# Autodesk Inventor assembly: Lath
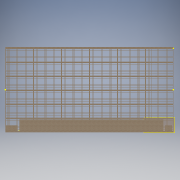
[picture p0: Inventor's stored thumbnail of the model, 180x180]
Saved by Autodesk Inventor 2018 (Build 220112000, 112)
## iProperties
Created: 2019-05-10
Part Number: Lath
Document SubType Name: Assembly
Designer: 10043883
Author: 10043883
## Documents named in this file (5)
- C:\Users\10043883\Documents\GitHub\IED-files\Lathhouse\Lath.iam
- C:\Users\10043883\Documents\GitHub\IED-files\Lathhouse\Lathhouse wall.ipt
- C:\Users\10043883\Documents\GitHub\IED-files\Lathhouse\Foor.ipt
- C:\Users\10043883\Documents\GitHub\IED-files\Lathhouse\Lathhouse roof.ipt
- C:\Users\10043883\Documents\GitHub\IED-files\Lathhouse\Front door.ipt
## Components (5 placed, 4 different names)
1. Foor:1 — Mate:13
2. Lathhouse wall:1 — Mate:11, Mate:12
3. Lathhouse roof:1 — Mate:9, Mate:11
4. Front door:1 — Mate:9
5. Front door:2 — Mate:12, Mate:13
## Relationships (4: Mate 4)
- Mate:9: Lathhouse roof:1 ↔ Front door:1
- Mate:11: Lathhouse wall:1 ↔ Lathhouse roof:1
- Mate:12: Lathhouse wall:1 ↔ Front door:2
- Mate:13: Foor:1 ↔ Front door:2
